# Autodesk Inventor assembly: złożenie2
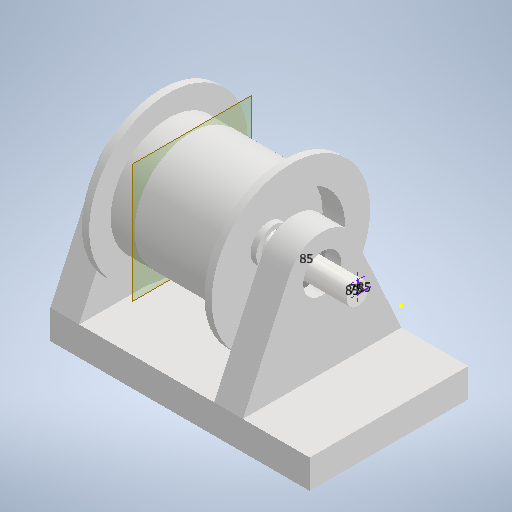
[picture p0: Inventor's stored thumbnail of the model, 512x512]
Saved by Autodesk Inventor 2025.2 (Build 292293000, 293)
## iProperties
Created: 2025-05-18
Part Number: złożenie2
Document SubType Name: Assembly
Designer: PC
Author: PC
## Documents named in this file (7)
- D:\Podstawy-Konstrukcji-Maszyn\Projekt3_temat3\src\Assemblies\złożenie2.iam
- D:\Podstawy-Konstrukcji-Maszyn\Projekt3_temat3\src\Parts\Wał4.ipt
- D:\Podstawy-Konstrukcji-Maszyn\Projekt3_temat3\src\Parts\1415151513515.ipt
- D:\Podstawy-Konstrukcji-Maszyn\Projekt3_temat3\src\ContentCenter\pl-PL\BS 290 SKF(05)\BS 290 SKF - SKF QJ 230 N2.ipt
- D:\Podstawy-Konstrukcji-Maszyn\Projekt3_temat3\src\Assemblies\Połączenie wpustowe1.iam
- D:\Podstawy-Konstrukcji-Maszyn\Projekt3_temat3\src\Assemblies\Połączenie wpustowe2.iam
- D:\Podstawy-Konstrukcji-Maszyn\Projekt3_temat3\src\Parts\podstawa.ipt
## Components (7 placed, 5 different names)
1. Wał:1 — Równoległe:1, Zestawiające:4, Kątowe:3, Kątowe:5, Równoległe:5, Kątowe:7, Zestawiające:7, Równoległe:6, Kątowe:8, Zestawiające:8, Kątowe:9
2. 1415151513515:1 — Zestawiające:4, Kątowe:3, Kątowe:5, Kątowe:9
3. BS 290 SKF- do styku czteropunktowego SKF QJ 230 N2:1
4. BS 290 SKF- do styku czteropunktowego SKF QJ 230 N2:2 — Walcowe:1
5. Połączenie wpustowe:1 [sub-assembly] — Równoległe:5, Kątowe:7, Zestawiające:7
6. Połączenie wpustowe:2 [sub-assembly] — Równoległe:6, Kątowe:8, Zestawiające:8
7. podstawa:1 — Walcowe:1
## Relationships (13: Angle 5, Flush 4, Mate 3, CylindricalJoint 1)
- Równoległe:1 [Flush]: Wał:1
- Równoległe:2 [Flush] (-200 mm)
- Zestawiające:4 [Mate] (180 mm): Wał:1 ↔ 1415151513515:1
- Kątowe:3 [Angle] (90 deg): Wał:1 ↔ 1415151513515:1
- Kątowe:5 [Angle] (90 deg): Wał:1 ↔ 1415151513515:1
- Równoległe:5 [Flush] (204.9231 mm): Wał:1 ↔ Połączenie wpustowe:1
- Kątowe:7 [Angle] (180 deg): Wał:1 ↔ Połączenie wpustowe:1
- Zestawiające:7 [Mate]: Wał:1 ↔ Połączenie wpustowe:1
- Równoległe:6 [Flush] (204.9722 mm): Wał:1 ↔ Połączenie wpustowe:2
- Kątowe:8 [Angle] (0 deg): Wał:1 ↔ Połączenie wpustowe:2
- Zestawiające:8 [Mate]: Wał:1 ↔ Połączenie wpustowe:2
- Kątowe:9 [Angle] (90 deg): Wał:1 ↔ 1415151513515:1
- Walcowe:1 [CylindricalJoint]: BS 290 SKF- do styku czteropunktowego SKF QJ 230 N2:2 ↔ podstawa:1
